# Autodesk Inventor assembly: yaw roll propuesta
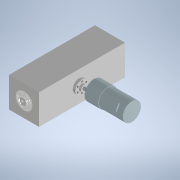
[picture p0: Inventor's stored thumbnail of the model, 180x180]
Saved by Autodesk Inventor 2020.3 (Build 243373000, 373)
## iProperties
Created: 2021-01-22
Part Number: yaw roll propuesta
Document SubType Name: Assembly
Designer: Yu Jinyu
Author: Yu Jinyu
## Documents named in this file (6)
- C:\Users\Yu Jinyu\OneDrive\Escritorio\Yaw Roll Nuevo\yaw roll propuesta.iam
- C:\Users\Yu Jinyu\OneDrive\Escritorio\Yaw Roll Nuevo\Motor Banebot.iam
- C:\Users\Yu Jinyu\OneDrive\Escritorio\Yaw Roll Nuevo\banebot soporte.ipt
- C:\Users\Yu Jinyu\OneDrive\Escritorio\Yaw Roll Nuevo\rodamientov2.ipt
- C:\Users\Yu Jinyu\OneDrive\Escritorio\Yaw Roll Nuevo\hub polulu.ipt
- C:\Users\Yu Jinyu\OneDrive\Escritorio\Yaw Roll Nuevo\Pololu37D.ipt
## Components (5 placed, 5 different names)
1. Motor Banebot:1 [sub-assembly] — Insert:2
2. banebot soporte:1 — Insert:1, Mate:1
3. rodamientov2:1 — Insert:1, Insert:2
4. hub polulu:1 — Mate:1, Insert:3
5. Pololu37D:2 — Insert:3
## Relationships (4: Insert 3, Mate 1)
- Insert:1 (-8 mm): banebot soporte:1 ↔ rodamientov2:1
- Insert:2 (78 mm): Motor Banebot:1 ↔ rodamientov2:1
- Mate:1: banebot soporte:1 ↔ hub polulu:1
- Insert:3 (-9 mm): hub polulu:1 ↔ Pololu37D:2
